# Autodesk Inventor assembly: 膝_6_1_MIR
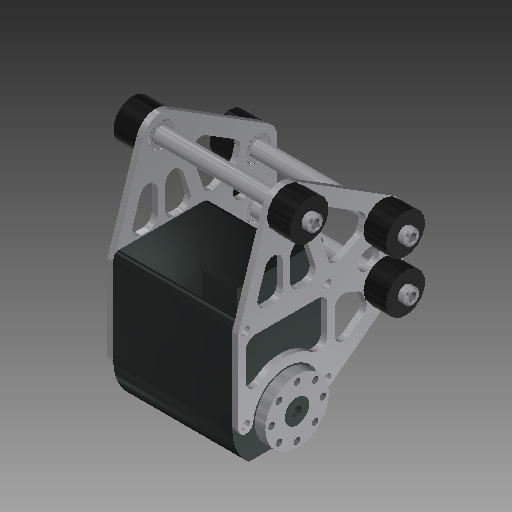
[picture p0: Inventor's stored thumbnail of the model, 512x512]
Saved by Autodesk Inventor 2018 (Build 220112000, 112)
## iProperties
Created: 2018-10-12
Part Number: 膝_6_1_MIR
Material: 一般
Document SubType Name: Assembly
Designer: taka
Mass: 161.264 g
Surface Area: 303.787 cm^2
Volume: 72.1671 cm^3
Density: 2.23459 g/cm^3
Author: taka
## Documents named in this file (7)
- C:\Users\taka\Documents\github\OpenPlatform\mechanism\OpenPlatform_ver3_0\下半身_160823\膝\膝_6_1_MIR.iam
- C:\Users\taka\Documents\github\OpenPlatform\mechanism\OpenPlatform_ver3_0\既製品\B3M11xx.ipt
- C:\Users\taka\Documents\github\OpenPlatform\mechanism\OpenPlatform_ver3_0\下半身_160823\膝\膝_メインフレーム.ipt
- C:\Users\taka\Documents\github\OpenPlatform\mechanism\OpenPlatform_ver3_0\既製品\SETF5-63_5-M3-N3.ipt
- C:\Users\taka\Documents\github\OpenPlatform\mechanism\OpenPlatform_ver3_0\既製品\NSK_RB_MF85ZZ\MF85ZZ.iam
- C:\Users\taka\Documents\github\OpenPlatform\mechanism\OpenPlatform_ver3_0\既製品\free_horn.ipt
- C:\Users\taka\Documents\github\OpenPlatform\mechanism\OpenPlatform_ver3_0\下半身\リンク\スペーサ\膝_同軸_スペーサ_1_5.ipt
## Components (19 placed, 6 different names)
1. B3M11xx:1 — 挿入:18, 挿入:19, 挿入:20, 挿入:21
2. 膝_メインフレーム:1 — 挿入:18, 挿入:19
3. 膝_メインフレーム:2 — 挿入:20, 挿入:21
4. SETF5-63_5-M3-N3:1 — 挿入:23
5. MF85ZZ:1 [sub-assembly]
6. MF85ZZ:2 [sub-assembly]
7. MF85ZZ:3 [sub-assembly]
8. MF85ZZ:4 [sub-assembly]
9. MF85ZZ:5 [sub-assembly]
10. MF85ZZ:6 [sub-assembly]
11. SETF5-63_5-M3-N3:2 — 挿入:24
12. SETF5-63_5-M3-N3:3 — 挿入:22
13. free_horn:1
14. 膝_同軸_スペーサ_1_5:1
15. 膝_同軸_スペーサ_1_5:2
16. 膝_同軸_スペーサ_1_5:3
17. 膝_同軸_スペーサ_1_5:4 — 挿入:22
18. 膝_同軸_スペーサ_1_5:5 — 挿入:23
19. 膝_同軸_スペーサ_1_5:6 — 挿入:24
## Relationships (20: Insert 20)
- [Insert]: 膝_メインフレーム:2 ↔ MF85ZZ:4
- [Insert]: 膝_メインフレーム:2 ↔ MF85ZZ:5
- [Insert]: 膝_メインフレーム:2 ↔ MF85ZZ:6
- [Insert]: 膝_メインフレーム:1 ↔ MF85ZZ:1
- [Insert]: 膝_メインフレーム:1 ↔ MF85ZZ:3
- [Insert]: 膝_メインフレーム:1 ↔ MF85ZZ:2
- [Insert]: B3M11xx:1 ↔ free_horn:1
- [Insert]: MF85ZZ:1 ↔ 膝_同軸_スペーサ_1_5:3
- [Insert]: MF85ZZ:3 ↔ 膝_同軸_スペーサ_1_5:2
- [Insert]: MF85ZZ:2 ↔ 膝_同軸_スペーサ_1_5:1
- [Insert]: MF85ZZ:6 ↔ 膝_同軸_スペーサ_1_5:4
- [Insert]: MF85ZZ:5 ↔ 膝_同軸_スペーサ_1_5:5
- [Insert]: MF85ZZ:4 ↔ 膝_同軸_スペーサ_1_5:6
- 挿入:18 [Insert]: B3M11xx:1 ↔ 膝_メインフレーム:1
- 挿入:19 [Insert]: B3M11xx:1 ↔ 膝_メインフレーム:1
- 挿入:20 [Insert]: B3M11xx:1 ↔ 膝_メインフレーム:2
- 挿入:21 [Insert]: B3M11xx:1 ↔ 膝_メインフレーム:2
- 挿入:22 [Insert] (-2.5 mm): SETF5-63_5-M3-N3:3 ↔ 膝_同軸_スペーサ_1_5:4
- 挿入:23 [Insert] (-2.5 mm): SETF5-63_5-M3-N3:1 ↔ 膝_同軸_スペーサ_1_5:5
- 挿入:24 [Insert] (-2.5 mm): SETF5-63_5-M3-N3:2 ↔ 膝_同軸_スペーサ_1_5:6
